# Autodesk Inventor assembly: 12_outer_carriage_with_cable_pass_trough
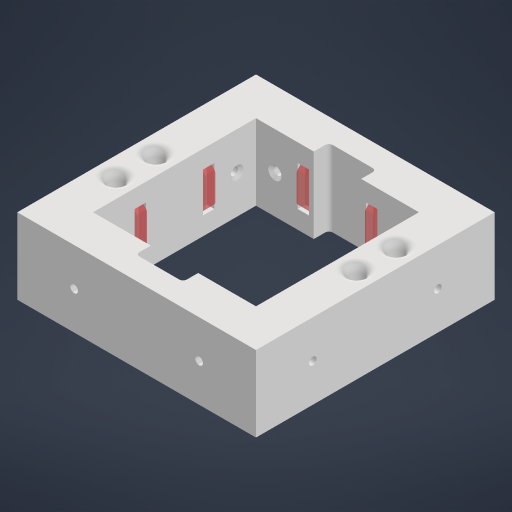
[picture p0: Inventor's stored thumbnail of the model, 512x512]
Saved by Autodesk Inventor 2024 (Build 280153000, 153)
## iProperties
Created: 2023-05-24
Part Number: 12_outer_carriage_with_cable_pass_trough
Document SubType Name: Assembly
Designer: aasmu
Author: aasmu
## Documents named in this file (4)
- C:\Users\aasmu\Documents\standing_desk\outer_glide_carriage\12_outer_carriage_with_cable_pass_trough.iam
- C:\Users\aasmu\Documents\standing_desk\outer_glide_carriage\03_one_side_with_outer_cabel_pass_trough.ipt
- C:\Users\aasmu\Documents\standing_desk\outer_glide_carriage\04_one_side_for_with_inner_cabel_pass_trough.ipt
- C:\Users\aasmu\Documents\standing_desk\inner_glide_carriage\04_steal_glide_plate.ipt
## Components (12 placed, 3 different names)
1. 03_one_side_with_outer_cabel_pass_trough:1 — Rigid:1, Rigid:10, Rigid:11
2. 03_one_side_with_outer_cabel_pass_trough:2 — Rigid:2, Rigid:3, Rigid:6, Rigid:7
3. 04_one_side_for_with_inner_cabel_pass_trough:1 — Rigid:1, Rigid:2, Rigid:8, Rigid:9
4. 04_one_side_for_with_inner_cabel_pass_trough:2 — Rigid:3, Rigid:4, Rigid:5
5. 04_steal_glide_plate:1 — Rigid:5
6. 04_steal_glide_plate:2 — Rigid:4
7. 04_steal_glide_plate:3 — Rigid:6
8. 04_steal_glide_plate:4 — Rigid:7
9. 04_steal_glide_plate:5 — Rigid:8
10. 04_steal_glide_plate:6 — Rigid:9
11. 04_steal_glide_plate:7 — Rigid:10
12. 04_steal_glide_plate:8 — Rigid:11
## Relationships (11: WeldJoint 11)
- Rigid:1 [WeldJoint]: 03_one_side_with_outer_cabel_pass_trough:1 ↔ 04_one_side_for_with_inner_cabel_pass_trough:1
- Rigid:2 [WeldJoint]: 03_one_side_with_outer_cabel_pass_trough:2 ↔ 04_one_side_for_with_inner_cabel_pass_trough:1
- Rigid:3 [WeldJoint]: 03_one_side_with_outer_cabel_pass_trough:2 ↔ 04_one_side_for_with_inner_cabel_pass_trough:2
- Rigid:4 [WeldJoint]: 04_one_side_for_with_inner_cabel_pass_trough:2 ↔ 04_steal_glide_plate:2
- Rigid:5 [WeldJoint]: 04_one_side_for_with_inner_cabel_pass_trough:2 ↔ 04_steal_glide_plate:1
- Rigid:6 [WeldJoint]: 03_one_side_with_outer_cabel_pass_trough:2 ↔ 04_steal_glide_plate:3
- Rigid:7 [WeldJoint]: 03_one_side_with_outer_cabel_pass_trough:2 ↔ 04_steal_glide_plate:4
- Rigid:8 [WeldJoint]: 04_one_side_for_with_inner_cabel_pass_trough:1 ↔ 04_steal_glide_plate:5
- Rigid:9 [WeldJoint]: 04_one_side_for_with_inner_cabel_pass_trough:1 ↔ 04_steal_glide_plate:6
- Rigid:10 [WeldJoint]: 03_one_side_with_outer_cabel_pass_trough:1 ↔ 04_steal_glide_plate:7
- Rigid:11 [WeldJoint]: 03_one_side_with_outer_cabel_pass_trough:1 ↔ 04_steal_glide_plate:8
